# Autodesk Inventor assembly: 9P Sprocket
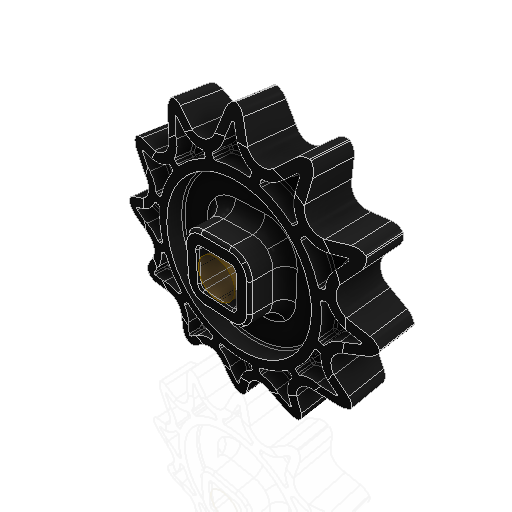
[picture p0: Inventor's stored thumbnail of the model, 512x512]
Saved by Autodesk Inventor 2025.2 (Build 292293000, 293)
## iProperties
Created: 2022-08-02
Part Number: 9P Sprocket
Document SubType Name: Assembly
Designer: ylu12
Author: ylu12
## Documents named in this file (3)
- C:\Users\avere\VEX-CAD\ROBOPROS-CAD-Inventor\Motion\Sprockets\9P Sprocket\9P 12T Sprocket, No Insert.iam
- C:\Users\avere\VEX-CAD\ROBOPROS-CAD-Inventor\Motion\Sprockets\Reference Files\9P 12T Sprocket, No Insert.ipt
- C:\Users\avere\VEX-CAD\ROBOPROS-CAD-Inventor\Motion\Sprockets\9P Sprocket.iam
## Components (1 placed, 1 different names)
1. 12T — Mate:7, Mate:8, Flush:4
## Relationships (3: Mate 2, Flush 1)
- Mate:7: 12T
- Mate:8: 12T
- Flush:4: 12T
